# Autodesk Inventor assembly: Display_Unit
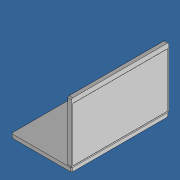
[picture p0: Inventor's stored thumbnail of the model, 180x180]
Saved by Autodesk Inventor 2020 (Build 240168000, 168)
## iProperties
Created: 2021-04-28
Part Number: Display_Unit
Document SubType Name: Assembly
Designer: ken113
Author: ken113
## Documents named in this file (2)
- D:\Document\Github\Eto_Project\Hardware\Asem\Display_Unit.iam
- D:\Document\Github\Eto_Project\Hardware\Parts\Display\Display.ipt
## Components (2 placed, 1 different names)
1. Display:1 — メイト:1, フラッシュ:1, フラッシュ:2
2. Display:2 — メイト:1, フラッシュ:1, フラッシュ:2
## Relationships (3: Flush 2, Mate 1)
- メイト:1 [Mate]: Display:1 ↔ Display:2
- フラッシュ:1 [Flush]: Display:1 ↔ Display:2
- フラッシュ:2 [Flush]: Display:1 ↔ Display:2
